# Autodesk Inventor assembly: Asem
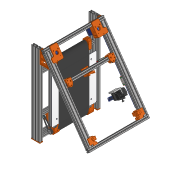
[picture p0: Inventor's stored thumbnail of the model, 180x180]
Saved by Autodesk Inventor 2020.1 (Build 241239000, 239)
## iProperties
Created: 2020-10-05
Part Number: Asem
Document SubType Name: Assembly
Designer: magnarecta
Author: magnarecta
## Documents named in this file (7)
- D:\ken113\Documents\GitHub\Cheap_Belt_Printer\Model\Asem\Asem.iam
- D:\ken113\Documents\GitHub\Cheap_Belt_Printer\Model\Asem\CoreXY_Unit_Asem.iam
- D:\ken113\Documents\GitHub\Cheap_Belt_Printer\Model\Asem\Belt_Unit_Asem_Rev2.iam
- D:\ken113\Documents\GitHub\Cheap_Belt_Printer\Model\Parts\MISUMI\HFS5-2020-380_Autodesk_Inventor_2020_20201006 (1)\HFS5-2020-380.ipt
- D:\ken113\Documents\GitHub\Cheap_Belt_Printer\Model\Parts\MISUMI\HFS5-2060-560_Autodesk_Inventor_2020_20201006\HFS5-2060-560.ipt
- D:\ken113\Documents\GitHub\Cheap_Belt_Printer\Model\Parts\Print_Parts\Print_Parts_S.ipt
- D:\ken113\Documents\GitHub\Cheap_Belt_Printer\Model\Parts\Print_Parts\Print_Parts_U.ipt
## Components (12 placed, 6 different names)
1. CoreXY_Unit_Asem:1 [sub-assembly] — フラッシュ:13, フラッシュ:14, フラッシュ:22, メイト:10, メイト:12, メイト:13
2. Belt_Unit_Asem_Rev2:1 [sub-assembly] — フラッシュ:13, メイト:1, メイト:2
3. HFS5-2020-380:1 — メイト:2, フラッシュ:14, フラッシュ:15, フラッシュ:17, メイト:5, メイト:6
4. HFS5-2020-380:2 — メイト:1, フラッシュ:15
5. HFS5-2020-380:4 — メイト:3, メイト:4, フラッシュ:16, フラッシュ:17, フラッシュ:20, フラッシュ:21, メイト:7
6. HFS5-2060-560:1 — メイト:3, メイト:6, フラッシュ:18, フラッシュ:19, メイト:11, フラッシュ:23, フラッシュ:24, メイト:15, フラッシュ:25, フラッシュ:28
7. HFS5-2060-560:2 — メイト:4, フラッシュ:16, メイト:5, フラッシュ:18, フラッシュ:19, フラッシュ:20, メイト:8, メイト:9, メイト:14, フラッシュ:26, フラッシュ:27
8. HFS5-2020-380:5 — フラッシュ:21, メイト:7, メイト:8
9. Print_Parts_S:1 — メイト:9, フラッシュ:22, メイト:10
10. Print_Parts_S:2 — メイト:11, フラッシュ:23, メイト:12, メイト:13, フラッシュ:24
11. Print_Parts_U:1 — メイト:14, フラッシュ:26, フラッシュ:27
12. Print_Parts_U:2 — メイト:15, フラッシュ:25, フラッシュ:28
## Relationships (31: Flush 16, Mate 15)
- フラッシュ:13 [Flush] (-55 mm): CoreXY_Unit_Asem:1 ↔ Belt_Unit_Asem_Rev2:1
- メイト:1 [Mate]: Belt_Unit_Asem_Rev2:1 ↔ HFS5-2020-380:2
- メイト:2 [Mate]: Belt_Unit_Asem_Rev2:1 ↔ HFS5-2020-380:1
- フラッシュ:14 [Flush] (20 mm): CoreXY_Unit_Asem:1 ↔ HFS5-2020-380:1
- フラッシュ:15 [Flush]: HFS5-2020-380:1 ↔ HFS5-2020-380:2
- メイト:3 [Mate]: HFS5-2020-380:4 ↔ HFS5-2060-560:1
- メイト:4 [Mate]: HFS5-2020-380:4 ↔ HFS5-2060-560:2
- フラッシュ:16 [Flush] (20 mm): HFS5-2020-380:4 ↔ HFS5-2060-560:2
- フラッシュ:17 [Flush]: HFS5-2020-380:1 ↔ HFS5-2020-380:4
- メイト:5 [Mate]: HFS5-2020-380:1 ↔ HFS5-2060-560:2
- メイト:6 [Mate]: HFS5-2020-380:1 ↔ HFS5-2060-560:1
- フラッシュ:18 [Flush]: HFS5-2060-560:1 ↔ HFS5-2060-560:2
- フラッシュ:19 [Flush]: HFS5-2060-560:1 ↔ HFS5-2060-560:2
- フラッシュ:20 [Flush]: HFS5-2020-380:4 ↔ HFS5-2060-560:2
- フラッシュ:21 [Flush]: HFS5-2020-380:4 ↔ HFS5-2020-380:5
- メイト:7 [Mate]: HFS5-2020-380:4 ↔ HFS5-2020-380:5
- メイト:8 [Mate]: HFS5-2060-560:2 ↔ HFS5-2020-380:5
- メイト:9 [Mate]: HFS5-2060-560:2 ↔ Print_Parts_S:1
- フラッシュ:22 [Flush]: CoreXY_Unit_Asem:1 ↔ Print_Parts_S:1
- メイト:10 [Mate]: CoreXY_Unit_Asem:1 ↔ Print_Parts_S:1
- メイト:11 [Mate]: HFS5-2060-560:1 ↔ Print_Parts_S:2
- フラッシュ:23 [Flush]: HFS5-2060-560:1 ↔ Print_Parts_S:2
- メイト:12 [Mate]: CoreXY_Unit_Asem:1 ↔ Print_Parts_S:2
- メイト:13 [Mate]: CoreXY_Unit_Asem:1 ↔ Print_Parts_S:2
- フラッシュ:24 [Flush]: HFS5-2060-560:1 ↔ Print_Parts_S:2
- メイト:14 [Mate]: HFS5-2060-560:2 ↔ Print_Parts_U:1
- メイト:15 [Mate]: HFS5-2060-560:1 ↔ Print_Parts_U:2
- フラッシュ:25 [Flush]: HFS5-2060-560:1 ↔ Print_Parts_U:2
- フラッシュ:26 [Flush]: HFS5-2060-560:2 ↔ Print_Parts_U:1
- フラッシュ:27 [Flush]: HFS5-2060-560:2 ↔ Print_Parts_U:1
- フラッシュ:28 [Flush]: HFS5-2060-560:1 ↔ Print_Parts_U:2
